# Autodesk Inventor assembly: B30037
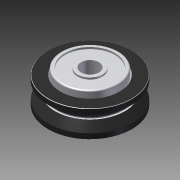
[picture p0: Inventor's stored thumbnail of the model, 180x180]
Saved by Autodesk Inventor 2014 (Build 180170000, 170)
## iProperties
Created: 2012-01-16
Part Number: B30037
Document SubType Name: Assembly
Designer: ERF
Description: Dual Bearing V Wheel Kit (assembly)
Mass: 3.05191 g
Surface Area: 39.551 cm^2
Volume: 2.4421 cm^3
Density: 1.24971 g/cm^3
Vendor: custom
Stock Number: B30037_ASM
Author: ERF
## Documents named in this file (4)
- C:\Users\Edward\Desktop\Shapeoko_v2.0\B30037.iam
- C:\Users\Edward\Desktop\Shapeoko_v2.0\B17021.ipt
- C:\Users\Edward\Desktop\Shapeoko_v2.0\BEARING_5_16_5.ipt
- C:\Users\Edward\Desktop\Shapeoko_v2.0\B18026.ipt
## Components (4 placed, 3 different names)
1. B17021:1 — Insert:1, Insert:3
2. BEARING_5_16_5:1 — Insert:3
3. B18026:1 — Insert:4
4. BEARING_5_16_5:2 — Insert:1, Insert:4
## Relationships (3: Insert 3)
- Insert:1: B17021:1 ↔ BEARING_5_16_5:2
- Insert:3: B17021:1 ↔ BEARING_5_16_5:1
- Insert:4: B18026:1 ↔ BEARING_5_16_5:2
